# Autodesk Inventor assembly: liftidea1
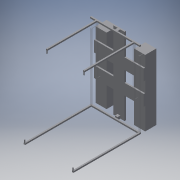
[picture p0: Inventor's stored thumbnail of the model, 180x180]
Saved by Autodesk Inventor 2017 (Build 210142000, 142)
## iProperties
Created: 2017-05-30
Part Number: liftidea1
Document SubType Name: Assembly
Designer: User
Author: User
## Documents named in this file (8)
- C:\Robotics\CAD\2016-17_CAD\liftidea1.iam
- C:\Robotics\CAD\2016-17_CAD\topbarlift.ipt
- C:\Robotics\CAD\2016-17_CAD\backplatelift.ipt
- C:\Robotics\CAD\2016-17_CAD\bottombarlift.ipt
- C:\Robotics\CAD\2016-17_CAD\bottombarliftconnector.ipt
- C:\Robotics\CAD\2016-17_CAD\halfinchspacer.ipt
- C:\Robotics\CAD\2016-17_CAD\outlineslides.ipt
- C:\Robotics\CAD\2016-17_CAD\capballgripperbar.ipt
## Components (23 placed, 7 different names)
1. topbarlift:1 — Mate:1, Flush:1, Flush:2, Flush:27, Mate:18, Flush:33, Flush:34
2. topbarlift:2 — Mate:2, Flush:3, Flush:4, Flush:30, Mate:17, Flush:31, Flush:32
3. backplatelift:1 — Flush:5, Flush:7, Mate:7, Flush:13, Flush:14, Mate:9, Flush:15, Flush:16, Mate:11, Flush:17, Flush:18, Mate:12, Flush:19, Flush:20, Flush:21, Flush:22
4. bottombarlift:1 — Mate:6, Flush:11, Flush:12, Mate:19, Flush:35, Flush:36
5. bottombarlift:2 — Mate:5, Flush:9, Flush:10, Mate:20, Flush:37, Flush:38
6. topbarlift:3 — Mate:1, Flush:1, Flush:2, Mate:2, Flush:3, Flush:4, Flush:5, Mate:8, Flush:21, Mate:15, Flush:28, Mate:16, Flush:29
7. bottombarliftconnector:1 — Flush:7, Mate:5, Flush:9, Flush:10, Mate:6, Flush:11, Flush:12, Mate:10, Flush:22, Mate:13, Flush:23, Flush:24, Mate:14, Flush:25, Flush:26
8. halfinchspacer:1 — Mate:9, Flush:15, Mate:10, Flush:16
9. halfinchspacer:2 — Mate:7, Flush:13, Mate:8, Flush:14
10. outlineslides:1 — Mate:11, Flush:17, Flush:18
11. outlineslides:2 — Mate:12, Flush:19, Flush:20
12. bottombarlift:3 — Mate:14, Flush:25, Flush:26, Flush:39, Flush:40, Mate:22
13. bottombarlift:4 — Mate:13, Flush:23, Flush:24, Flush:41, Flush:42, Mate:23, Mate:24
14. topbarlift:4 — Mate:15, Flush:27, Flush:28, Flush:45, Flush:46, Mate:21
15. topbarlift:5 — Mate:16, Flush:29, Flush:30, Flush:43, Flush:44
16. capballgripperbar:1 — Mate:17, Flush:31, Flush:32
17. capballgripperbar:2 — Mate:20, Flush:37, Flush:38
18. capballgripperbar:3 — Mate:19, Flush:35, Flush:36
19. capballgripperbar:4 — Mate:18, Flush:33, Flush:34
20. capballgripperbar:5 — Flush:43, Flush:44, Mate:23
21. capballgripperbar:6 — Flush:41, Flush:42, Mate:24
22. capballgripperbar:7 — Flush:45, Flush:46, Mate:21
23. capballgripperbar:8 — Flush:39, Flush:40, Mate:22
## Relationships (66: Flush 44, Mate 22)
- Mate:1: topbarlift:1 ↔ topbarlift:3
- Flush:1 (-25.4 mm): topbarlift:1 ↔ topbarlift:3
- Flush:2: topbarlift:1 ↔ topbarlift:3
- Mate:2: topbarlift:2 ↔ topbarlift:3
- Flush:3 (25.4 mm): topbarlift:2 ↔ topbarlift:3
- Flush:4: topbarlift:2 ↔ topbarlift:3
- Flush:5: backplatelift:1 ↔ topbarlift:3
- Flush:7: backplatelift:1 ↔ bottombarliftconnector:1
- Mate:5: bottombarlift:2 ↔ bottombarliftconnector:1
- Flush:9: bottombarlift:2 ↔ bottombarliftconnector:1
- Flush:10: bottombarlift:2 ↔ bottombarliftconnector:1
- Mate:6: bottombarlift:1 ↔ bottombarliftconnector:1
- Flush:11: bottombarlift:1 ↔ bottombarliftconnector:1
- Flush:12: bottombarlift:1 ↔ bottombarliftconnector:1
- Mate:7: backplatelift:1 ↔ halfinchspacer:2
- Flush:13: backplatelift:1 ↔ halfinchspacer:2
- Mate:8: topbarlift:3 ↔ halfinchspacer:2
- Flush:14 (19.05 mm): backplatelift:1 ↔ halfinchspacer:2
- Mate:9: backplatelift:1 ↔ halfinchspacer:1
- Flush:15: backplatelift:1 ↔ halfinchspacer:1
- Mate:10: bottombarliftconnector:1 ↔ halfinchspacer:1
- Flush:16 (19.05 mm): backplatelift:1 ↔ halfinchspacer:1
- Mate:11: backplatelift:1 ↔ outlineslides:1
- Flush:17: backplatelift:1 ↔ outlineslides:1
- Flush:18: backplatelift:1 ↔ outlineslides:1
- Mate:12: backplatelift:1 ↔ outlineslides:2
- Flush:19: backplatelift:1 ↔ outlineslides:2
- Flush:20: backplatelift:1 ↔ outlineslides:2
- Flush:21 (88.9 mm): backplatelift:1 ↔ topbarlift:3
- Flush:22 (88.9 mm): backplatelift:1 ↔ bottombarliftconnector:1
- Mate:13: bottombarliftconnector:1 ↔ bottombarlift:4
- Flush:23: bottombarliftconnector:1 ↔ bottombarlift:4
- Flush:24: bottombarliftconnector:1 ↔ bottombarlift:4
- Mate:14: bottombarliftconnector:1 ↔ bottombarlift:3
- Flush:25: bottombarliftconnector:1 ↔ bottombarlift:3
- Flush:26: bottombarliftconnector:1 ↔ bottombarlift:3
- Mate:15: topbarlift:3 ↔ topbarlift:4
- Flush:27: topbarlift:1 ↔ topbarlift:4
- Flush:28: topbarlift:3 ↔ topbarlift:4
- Mate:16: topbarlift:3 ↔ topbarlift:5
- Flush:29: topbarlift:3 ↔ topbarlift:5
- Flush:30: topbarlift:2 ↔ topbarlift:5
- Mate:17: topbarlift:2 ↔ capballgripperbar:1
- Flush:31: topbarlift:2 ↔ capballgripperbar:1
- Flush:32 (1.5875 mm): topbarlift:2 ↔ capballgripperbar:1
- Mate:18: topbarlift:1 ↔ capballgripperbar:4
- Flush:33: topbarlift:1 ↔ capballgripperbar:4
- Flush:34 (1.5875 mm): topbarlift:1 ↔ capballgripperbar:4
- Mate:19: bottombarlift:1 ↔ capballgripperbar:3
- Flush:35: bottombarlift:1 ↔ capballgripperbar:3
- Flush:36 (1.5875 mm): bottombarlift:1 ↔ capballgripperbar:3
- Mate:20: bottombarlift:2 ↔ capballgripperbar:2
- Flush:37: bottombarlift:2 ↔ capballgripperbar:2
- Flush:38 (1.5875 mm): bottombarlift:2 ↔ capballgripperbar:2
- Flush:39: bottombarlift:3 ↔ capballgripperbar:8
- Flush:40 (1.5875 mm): bottombarlift:3 ↔ capballgripperbar:8
- Flush:41: bottombarlift:4 ↔ capballgripperbar:6
- Flush:42 (1.5875 mm): bottombarlift:4 ↔ capballgripperbar:6
- Flush:43 (1.5875 mm): topbarlift:5 ↔ capballgripperbar:5
- Flush:44: topbarlift:5 ↔ capballgripperbar:5
- Flush:45: topbarlift:4 ↔ capballgripperbar:7
- Flush:46 (1.5875 mm): topbarlift:4 ↔ capballgripperbar:7
- Mate:21: topbarlift:4 ↔ capballgripperbar:7
- Mate:22: bottombarlift:3 ↔ capballgripperbar:8
- Mate:23: bottombarlift:4 ↔ capballgripperbar:5
- Mate:24: bottombarlift:4 ↔ capballgripperbar:6
